# Autodesk Inventor assembly: sleds
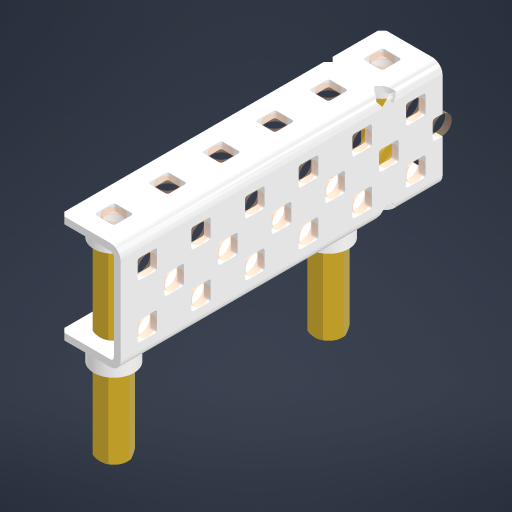
[picture p0: Inventor's stored thumbnail of the model, 512x512]
Saved by Autodesk Inventor 2023 (Build 270158000, 158)
## iProperties
Created: 2023-08-07
Part Number: sleds
Document SubType Name: Assembly
Designer: srbel
Author: srbel
## Documents named in this file (6)
- C:\CAD\OverUnderCAD\Drive\sleds.iam
- C:\CAD\OverUnderCAD\VEX-CAD-Inventor-1.4.0\Structure\C Channel\Aluminum 1x2x1\Alu C 1x2x1x6.ipt
- C:\CAD\OverUnderCAD\VEX-CAD-Inventor-1.4.0\Structure\Standoff\Standoff .75.ipt
- C:\CAD\OverUnderCAD\VEX-CAD-Inventor-1.4.0\Structure\Standoff.ipt
- C:\CAD\OverUnderCAD\VEX-CAD-Inventor-1.4.0\Motion\Spacers\Spacer Nylon .313 OD\NSpacer .313 OD x .125.ipt
- C:\CAD\OverUnderCAD\VEX-CAD-Inventor-1.4.0\Motion\Spacers\Spacer Nylon .313 OD.ipt
## Components (9 placed, 3 different names)
1. Alu C 1x2x1x6:1 — Insert:5, Insert:7, Insert:10, Insert:12
2. NSpacer .313 OD x .125:3 — Insert:5, Insert:6
3. Standoff .75:3 — Insert:6
4. NSpacer .313 OD x .125:4 — Insert:7, Insert:8
5. Standoff .75:4 — Insert:8
6. NSpacer .313 OD x .125:5 — Insert:10
7. Standoff .75:5
8. NSpacer .313 OD x .125:6 — Insert:12
9. Standoff .75:6
## Relationships (8: Insert 8)
- Insert:5: Alu C 1x2x1x6:1 ↔ NSpacer .313 OD x .125:3
- Insert:6: NSpacer .313 OD x .125:3 ↔ Standoff .75:3
- Insert:7: Alu C 1x2x1x6:1 ↔ NSpacer .313 OD x .125:4
- Insert:8: NSpacer .313 OD x .125:4 ↔ Standoff .75:4
- [Insert]: NSpacer .313 OD x .125:5 ↔ Standoff .75:5
- Insert:10 (1.5875 mm): Alu C 1x2x1x6:1 ↔ NSpacer .313 OD x .125:5
- [Insert]: NSpacer .313 OD x .125:6 ↔ Standoff .75:6
- Insert:12 (1.5875 mm): Alu C 1x2x1x6:1 ↔ NSpacer .313 OD x .125:6
## Named parameters: d8_d5 = 0 mm, d10_d8_d5 = 0 mm
